# Autodesk Inventor assembly: ABD_Version_0.1_leftleg
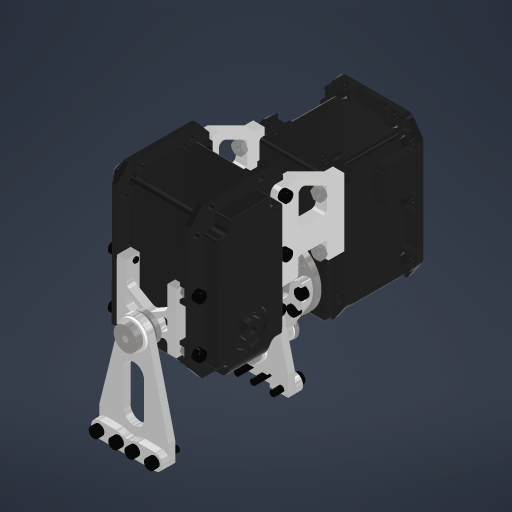
[picture p0: Inventor's stored thumbnail of the model, 512x512]
Saved by Autodesk Inventor 2024.3 (Build 283343000, 343)
## iProperties
Created: 2024-01-23
Part Number: ABD_Version_0.1_leftleg
Document SubType Name: Assembly
Designer: ASUS
Mass: 357.136 g
Surface Area: 604.848 cm^2
Volume: 181.423 cm^3
Density: 1.96853 g/cm^3
Author: ASUS
## Documents named in this file (14)
- C:\Users\ASUS\Desktop\test\v4_Frame_2025\ABD_V4_Left_OP.iam
- C:\Users\ASUS\Desktop\test\v4_Frame_2025\ABD_MX_64_Roll_Fixation_Set.iam
- C:\Users\ASUS\Desktop\test\v4_Frame_2025\Roll_Fixation_Frame_Back.ipt
- C:\Users\ASUS\Desktop\test\v4_Frame_2025\hip joint fix washer.ipt
- C:\Users\ASUS\Desktop\test\Screw_Set\hip_joint_fix_washer_10mm_Set.iam
- C:\Users\ASUS\Desktop\test\v4_Frame_2025\Front_Frame_Fixer_v2.iam
- C:\Users\ASUS\Desktop\test\ROBOTIS(Inventor 2024 ver.)\DXL\MX-64T.ipt
- C:\Users\ASUS\Desktop\test\v4_Frame_2025\Dynamixel Vertical fixation.ipt
- C:\Users\ASUS\Desktop\test\v4_Frame_2025\Dynamixel Vertical fixation_MIR.ipt
- C:\Users\ASUS\Desktop\test\v1_Frame\MISUMI\SLBNR2_5.ipt
- C:\Users\ASUS\Desktop\test\Screw_Set\Roll_Fixation_Frame_8mm_Set.iam
- C:\Users\ASUS\Desktop\test\Screw_Set\Roll_Fixation_Frame_8mm_Set_Backside.iam
- C:\Users\ASUS\Desktop\test\v4_Frame_2025\ABD_Slider_Set_v4.iam
- C:\Users\ASUS\Desktop\test\v4_Frame_2025\Crank_Fixation.iam
## Components (20 placed, 13 different names)
1. hip joint fix washer:1 — 메이트:50, 삽입:82, 메이트:64
2. hip joint fix washer:2 — 삽입:47, 메이트:29
3. hip_joint_fix_washer_10mm_Set:1 [sub-assembly] — 메이트:50, 메이트:64
4. hip_joint_fix_washer_10mm_Set:2 [sub-assembly] — 메이트:29, 메이트:43
5. Front_Frame_Fixer_v2:1 [sub-assembly] — 삽입:46, 삽입:81
6. ABD_MX_64_Roll_Fixation_Set:2 [sub-assembly] — 각도:3, 플러쉬:1, 삽입:46, 삽입:71, 메이트:45, 삽입:72, 메이트:46, 삽입:78
7. MX-64T:1 — 각도:3, 플러쉬:1, 메이트:36, 메이트:51, 메이트:52, 메이트:60, 각도:11, 메이트:61
8. Roll_Fixation_Frame_Back:3 — 삽입:47, 메이트:43, 삽입:79, 각도:11, 메이트:62, 메이트:63
9. Dynamixel Vertical fixation:2 — 메이트:47, 메이트:48, 메이트:51, 메이트:52
10. Dynamixel Vertical fixation_MIR:2 — 메이트:36, 메이트:58, 메이트:59, 메이트:60
11. SLBNR2_5:5
12. SLBNR2_5:6
13. SLBNR2_5:7
14. SLBNR2_5:8
15. Roll_Fixation_Frame_8mm_Set:1 [sub-assembly] — 삽입:71, 메이트:45
16. Roll_Fixation_Frame_8mm_Set_Backside:1 [sub-assembly] — 삽입:72, 메이트:46, 메이트:47, 메이트:48, 메이트:58, 메이트:59
17. Front_Frame_Fixer_v2:2 [sub-assembly] — 삽입:78, 삽입:79
18. ABD_Slider_Set_v4:1 [sub-assembly] — 메이트:61, 삽입:80
19. Crank_Fixation:1 [sub-assembly] — 삽입:80, 메이트:62, 메이트:63
20. Roll_Fixation_Frame_Back:4 — 삽입:81, 삽입:82
## Relationships (41: Mate 21, Insert 15, Angle 4, Flush 1)
- [Insert]: hip joint fix washer:1 ↔ hip_joint_fix_washer_10mm_Set:1
- [Mate]: hip joint fix washer:1 ↔ hip_joint_fix_washer_10mm_Set:1
- [Insert]: hip joint fix washer:2 ↔ hip_joint_fix_washer_10mm_Set:2
- [Mate]: hip joint fix washer:2 ↔ hip_joint_fix_washer_10mm_Set:2
- [Mate]: hip_joint_fix_washer_10mm_Set:1 ↔ hip_joint_fix_washer_10mm_Set:2
- [Mate]: hip_joint_fix_washer_10mm_Set:1 ↔ hip_joint_fix_washer_10mm_Set:2
- 각도:3 [Angle] (0 deg): ABD_MX_64_Roll_Fixation_Set:2 ↔ MX-64T:1
- 플러쉬:1 [Flush] (-3.1 mm): ABD_MX_64_Roll_Fixation_Set:2 ↔ MX-64T:1
- 삽입:46 [Insert]: Front_Frame_Fixer_v2:1 ↔ ABD_MX_64_Roll_Fixation_Set:2
- 삽입:47 [Insert]: hip joint fix washer:2 ↔ Roll_Fixation_Frame_Back:3
- 메이트:29 [Mate]: hip joint fix washer:2 ↔ hip_joint_fix_washer_10mm_Set:2
- [Insert]: Dynamixel Vertical fixation:2 ↔ SLBNR2_5:5
- [Insert]: Dynamixel Vertical fixation:2 ↔ SLBNR2_5:6
- [Insert]: Dynamixel Vertical fixation_MIR:2 ↔ SLBNR2_5:8
- [Insert]: Dynamixel Vertical fixation_MIR:2 ↔ SLBNR2_5:7
- [Angle] (0 deg): Dynamixel Vertical fixation_MIR:2 ↔ SLBNR2_5:7
- [Angle] (0 deg): Dynamixel Vertical fixation_MIR:2 ↔ SLBNR2_5:8
- 메이트:36 [Mate]: MX-64T:1 ↔ Dynamixel Vertical fixation_MIR:2
- 메이트:43 [Mate]: hip_joint_fix_washer_10mm_Set:2 ↔ Roll_Fixation_Frame_Back:3
- 삽입:71 [Insert]: ABD_MX_64_Roll_Fixation_Set:2 ↔ Roll_Fixation_Frame_8mm_Set:1
- 메이트:45 [Mate]: ABD_MX_64_Roll_Fixation_Set:2 ↔ Roll_Fixation_Frame_8mm_Set:1
- 삽입:72 [Insert]: ABD_MX_64_Roll_Fixation_Set:2 ↔ Roll_Fixation_Frame_8mm_Set_Backside:1
- 메이트:46 [Mate]: ABD_MX_64_Roll_Fixation_Set:2 ↔ Roll_Fixation_Frame_8mm_Set_Backside:1
- 메이트:47 [Mate]: Dynamixel Vertical fixation:2 ↔ Roll_Fixation_Frame_8mm_Set_Backside:1
- 메이트:48 [Mate]: Dynamixel Vertical fixation:2 ↔ Roll_Fixation_Frame_8mm_Set_Backside:1
- 메이트:50 [Mate]: hip joint fix washer:1 ↔ hip_joint_fix_washer_10mm_Set:1
- 삽입:78 [Insert]: ABD_MX_64_Roll_Fixation_Set:2 ↔ Front_Frame_Fixer_v2:2
- 삽입:79 [Insert]: Roll_Fixation_Frame_Back:3 ↔ Front_Frame_Fixer_v2:2
- 메이트:51 [Mate]: MX-64T:1 ↔ Dynamixel Vertical fixation:2
- 메이트:52 [Mate]: MX-64T:1 ↔ Dynamixel Vertical fixation:2
- 메이트:58 [Mate]: Dynamixel Vertical fixation_MIR:2 ↔ Roll_Fixation_Frame_8mm_Set_Backside:1
- 메이트:59 [Mate]: Dynamixel Vertical fixation_MIR:2 ↔ Roll_Fixation_Frame_8mm_Set_Backside:1
- 메이트:60 [Mate]: MX-64T:1 ↔ Dynamixel Vertical fixation_MIR:2
- 각도:11 [Angle] (0 deg): MX-64T:1 ↔ Roll_Fixation_Frame_Back:3
- 메이트:61 [Mate]: MX-64T:1 ↔ ABD_Slider_Set_v4:1
- 삽입:80 [Insert]: ABD_Slider_Set_v4:1 ↔ Crank_Fixation:1
- 메이트:62 [Mate]: Roll_Fixation_Frame_Back:3 ↔ Crank_Fixation:1
- 메이트:63 [Mate]: Roll_Fixation_Frame_Back:3 ↔ Crank_Fixation:1
- 삽입:81 [Insert]: Front_Frame_Fixer_v2:1 ↔ Roll_Fixation_Frame_Back:4
- 삽입:82 [Insert]: hip joint fix washer:1 ↔ Roll_Fixation_Frame_Back:4
- 메이트:64 [Mate]: hip joint fix washer:1 ↔ hip_joint_fix_washer_10mm_Set:1
## Named parameters: d1061_d1053 = 0 mm, d1062_d1054 = 0 mm, d1063_d1055 = 0 mm, d1064_d1056 = 0 mm, d1065_d1057 = 0 deg, d1066_d1058 = 0 deg
